# Autodesk Inventor assembly: hive
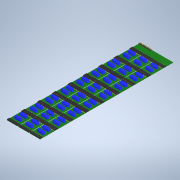
[picture p0: Inventor's stored thumbnail of the model, 180x180]
Saved by Autodesk Inventor 2021 (Build 250183000, 183)
## iProperties
Created: 2020-11-14
Part Number: hive
Document SubType Name: Assembly
Designer: Yatekii
Author: Yatekii
## Documents named in this file (3)
- C:\Users\Yatekii\repos\probe-rs\hive\mechanical\hive.iam
- C:\Users\Yatekii\repos\probe-rs\hive\mechanical\3lanes.iam
- C:\Users\Yatekii\repos\probe-rs\hive\mechanical\8channels.iam
## Components (49 placed, 2 different names)
1. 3lanes:1 [sub-assembly] — Rigid:1
2. 8channels:1 [sub-assembly] — Rigid:1
3. 8channels:2 [sub-assembly]
4. 8channels:3 [sub-assembly]
5. 8channels:4 [sub-assembly]
6. 8channels:5 [sub-assembly]
7. 8channels:6 [sub-assembly]
8. 8channels:7 [sub-assembly]
9. 8channels:8 [sub-assembly]
10. 8channels:9 [sub-assembly]
11. 8channels:10 [sub-assembly]
12. 8channels:11 [sub-assembly]
13. 8channels:12 [sub-assembly]
14. 8channels:13 [sub-assembly]
15. 8channels:14 [sub-assembly]
16. 8channels:15 [sub-assembly]
17. 8channels:16 [sub-assembly]
18. 8channels:17 [sub-assembly]
19. 8channels:18 [sub-assembly]
20. 8channels:19 [sub-assembly]
21. 8channels:20 [sub-assembly]
22. 8channels:21 [sub-assembly]
23. 8channels:22 [sub-assembly]
24. 8channels:23 [sub-assembly]
25. 8channels:24 [sub-assembly]
26. 8channels:25 [sub-assembly]
27. 8channels:26 [sub-assembly]
28. 8channels:27 [sub-assembly]
29. 8channels:28 [sub-assembly]
30. 8channels:29 [sub-assembly]
31. 8channels:30 [sub-assembly]
32. 8channels:31 [sub-assembly]
33. 8channels:32 [sub-assembly]
34. 8channels:33 [sub-assembly]
35. 8channels:34 [sub-assembly]
36. 8channels:35 [sub-assembly]
37. 8channels:36 [sub-assembly]
38. 8channels:37 [sub-assembly]
39. 8channels:38 [sub-assembly]
40. 8channels:39 [sub-assembly]
41. 8channels:40 [sub-assembly]
42. 8channels:41 [sub-assembly]
43. 8channels:42 [sub-assembly]
44. 8channels:43 [sub-assembly]
45. 8channels:44 [sub-assembly]
46. 8channels:45 [sub-assembly]
47. 8channels:46 [sub-assembly]
48. 8channels:47 [sub-assembly]
49. 8channels:48 [sub-assembly]
## Component patterns: (24 elements), (2 elements, first: 8channels:1), Component Pattern 1:2 (2 elements), Component Pattern 1:3 (2 elements), Component Pattern 1:4 (2 elements), Component Pattern 1:5 (2 elements), Component Pattern 1:6 (2 elements), Component Pattern 1:7 (2 elements), Component Pattern 1:8 (2 elements), Component Pattern 1:9 (2 elements), Component Pattern 1:10 (2 elements), Component Pattern 1:11 (2 elements), Component Pattern 1:12 (2 elements), Component Pattern 1:13 (2 elements), Component Pattern 1:14 (2 elements), Component Pattern 1:15 (2 elements), Component Pattern 1:16 (2 elements), Component Pattern 1:17 (2 elements), Component Pattern 1:18 (2 elements), Component Pattern 1:19 (2 elements), Component Pattern 1:20 (2 elements), Component Pattern 1:21 (2 elements), Component Pattern 1:22 (2 elements), Component Pattern 1:23 (2 elements), Component Pattern 1:24 (2 elements)
## Relationships (1: WeldJoint 1)
- Rigid:1 [WeldJoint] (0.5 mm): 3lanes:1 ↔ 8channels:1
